# Autodesk Inventor assembly: 8022581 ESBF-BS-40-100-16P---(0)
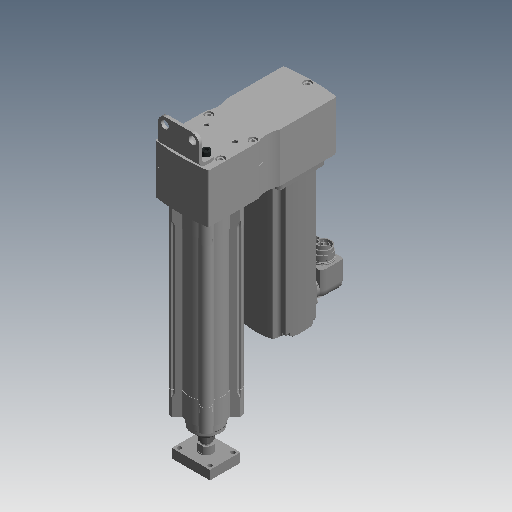
[picture p0: Inventor's stored thumbnail of the model, 512x512]
Saved by Autodesk Inventor 2021 (Build 250183000, 183)
## iProperties
Category: PARTsolutions
Company: FESTO
Part Number: 8022581 ESBF-BS-40-100-16P---(0)
Catalog Web Link: www.cadenas.de
Description: ESBF-Electro-cylinder
Vendor: FESTO
Document SubType Name: Assembly
Designer: partserver
Manufacturer: FESTO
Mass: 1707 g
Surface Area: 1273.02 cm^2
Volume: 500.946 cm^3
Density: 3.40756 g/cm^3
PSOL_IDENT_0: {ATYP=ASSISTANT},{DATA=script=$CADENAS_DATA/23d-libs/festo/webfesto.vbb&M_FAMILY=ESBF&M_GROUP=01&M_P
PSOL_IDENT_1: ARTNO=8022581&IDCODE1=ESBF-BS-40-100-16P&IDCODE2=&customer_number_cns=&MATES=1&LOD=HI&LOCKERP=0&SING
PSOL_IDENT_2: LEPART=1}
NB: 8022581 ESBF-BS-40-100-16P---(0)
NN: ESBF
NT: Electro-cylinder
NBSYN: $TNR. $TYP.---($HUBST.)
LINA: 8022581 ESBF-BS-40-100-16P
CATALOG: Festo
TNR: 8022581
TYP: ESBF-BS-40-100-16P
ANT: BS
KDM: 40
HUB: 100
SPI: 16P
HUBST: 0
AM: 24
WH: 29.5
L1: 14
L2: 244
L3: 18.4
L4: 14
L5: 3.3
L7: 24
L8: 4
G: 30
G1: 30
VA: 7
VD: 9
ZJ: 273.5
KK: M12x1.25
MM: 24
B: 39
D1: 24
D2: 8
D3: 40
BG: 16
EE: M7
E: 54
RT: M6
SW1: 13
SW2: 19
SW3: 6
TG: 38
CNSMASSEXACT: 1.707
SUPPLIER: FESTO
ARTICLENO: 8022581 ESBF-BS-40-100-16P---(0)
BOMINFO: 8022581 ESBF-BS-40-100-16P
CREATOR: CADENAS GmbH
Title: 8022581 ESBF-BS-40-100-16P
Author: Cadenas PARTsolutions
Comments: Electro-cylinder
## Documents named in this file (9)
- C:\Users\Santiago Suárez\Documents\GitHub\Dis.-Mecatronico-E6\Entrega Final\CAD\Mecanismo4dof\ActuadorAvance\AIS2021\8022581 ESBF-BS-40-100-16P---(0).iam
- C:\Users\Santiago Suárez\Documents\GitHub\Dis.-Mecatronico-E6\Entrega Final\CAD\Mecanismo4dof\ActuadorAvance\AIS2021\ESBF-BS-40-100---(ZR_-_-).ipt
- C:\Users\Santiago Suárez\Documents\GitHub\Dis.-Mecatronico-E6\Entrega Final\CAD\Mecanismo4dof\ActuadorAvance\AIS2021\ESBF-BS-40-100-5P---(KS_0).ipt
- C:\Users\Santiago Suárez\Documents\GitHub\Dis.-Mecatronico-E6\Entrega Final\CAD\Mecanismo4dof\ActuadorAvance\AIS2021\717739 GUK M10x0_75.ipt
- C:\Users\Santiago Suárez\Documents\GitHub\Dis.-Mecatronico-E6\Entrega Final\CAD\Mecanismo4dof\ActuadorAvance\AIS2021\ESBF-BS-40-ESBF-BS-40---(KSA).ipt
- C:\Users\Santiago Suárez\Documents\GitHub\Dis.-Mecatronico-E6\Entrega Final\CAD\Mecanismo4dof\ActuadorAvance\AIS2021\5242214 EMMT-AS-60-L-LS-RSB---(high).iam
- C:\Users\Santiago Suárez\Documents\GitHub\Dis.-Mecatronico-E6\Entrega Final\CAD\Mecanismo4dof\ActuadorAvance\36126 KSZ-M12x1,25.ipt
- C:\Users\Santiago Suárez\Documents\GitHub\Dis.-Mecatronico-E6\Entrega Final\CAD\Mecanismo4dof\ActuadorAvance\AIS2021\174370 HNC-40_(50).iam
- C:\Users\Santiago Suárez\Documents\GitHub\Dis.-Mecatronico-E6\Entrega Final\CAD\Mecanismo4dof\ActuadorAvance\AIS2021\2617488 EAMM-U-70-D40-60P-96.iam
## Components (8 placed, 8 different names)
1. ESBF-BS-40-100---(ZR_-_-):1 — KS_XY@1 <-> ANBAU_XY@2, KS_Z@1 <-> ANBAU_Z@2, KS_YZ@1 <-> ANBAU_YZ@2, GUA_XY@1 <-> ANBAU_XY@4, GUA_Z@1 <-> ANBAU_Z@4, GUA_YZ@1 <-> ANBAU_YZ@4, KSA_XY@1 <-> ANBAU_XY@5, KSA_Z@1 <-> ANBAU_Z@5, KSA_YZ@1 <-> ANBAU_YZ@5, Rigid:4
2. ESBF-BS-40-100-5P---(KS_0):1 — KS_XY@1 <-> ANBAU_XY@2, KS_Z@1 <-> ANBAU_Z@2, KS_YZ@1 <-> ANBAU_YZ@2, Rigid:2
3. 717739 GUK M10x0_75:1 — GUA_XY@1 <-> ANBAU_XY@4, GUA_Z@1 <-> ANBAU_Z@4, GUA_YZ@1 <-> ANBAU_YZ@4
4. ESBF-BS-40-ESBF-BS-40---(KSA):1 — KSA_XY@1 <-> ANBAU_XY@5, KSA_Z@1 <-> ANBAU_Z@5, KSA_YZ@1 <-> ANBAU_YZ@5
5. 5242214 EMMT-AS-60-L-LS-RSB---(high):1 [sub-assembly] — Rigid:3
6. 36126 KSZ-M12x1,25:1 — Rigid:2
7. 174370 HNC-40_(50):1 [sub-assembly] — Rigid:5
8. 2617488 EAMM-U-70-D40-60P-96:1 [sub-assembly] — Rigid:3, Rigid:4, Rigid:5
## Relationships (13: Mate 6, WeldJoint 4, Angle 3)
- KS_XY@1 <-> ANBAU_XY@2 [Mate]: ESBF-BS-40-100---(ZR_-_-):1 ↔ ESBF-BS-40-100-5P---(KS_0):1
- KS_Z@1 <-> ANBAU_Z@2 [Mate]: ESBF-BS-40-100---(ZR_-_-):1 ↔ ESBF-BS-40-100-5P---(KS_0):1
- KS_YZ@1 <-> ANBAU_YZ@2 [Angle] (0 deg): ESBF-BS-40-100---(ZR_-_-):1 ↔ ESBF-BS-40-100-5P---(KS_0):1
- GUA_XY@1 <-> ANBAU_XY@4 [Mate]: ESBF-BS-40-100---(ZR_-_-):1 ↔ 717739 GUK M10x0_75:1
- GUA_Z@1 <-> ANBAU_Z@4 [Mate]: ESBF-BS-40-100---(ZR_-_-):1 ↔ 717739 GUK M10x0_75:1
- GUA_YZ@1 <-> ANBAU_YZ@4 [Angle] (0 deg): ESBF-BS-40-100---(ZR_-_-):1 ↔ 717739 GUK M10x0_75:1
- KSA_XY@1 <-> ANBAU_XY@5 [Mate]: ESBF-BS-40-100---(ZR_-_-):1 ↔ ESBF-BS-40-ESBF-BS-40---(KSA):1
- KSA_Z@1 <-> ANBAU_Z@5 [Mate]: ESBF-BS-40-100---(ZR_-_-):1 ↔ ESBF-BS-40-ESBF-BS-40---(KSA):1
- KSA_YZ@1 <-> ANBAU_YZ@5 [Angle] (0 deg): ESBF-BS-40-100---(ZR_-_-):1 ↔ ESBF-BS-40-ESBF-BS-40---(KSA):1
- Rigid:2 [WeldJoint]: ESBF-BS-40-100-5P---(KS_0):1 ↔ 36126 KSZ-M12x1,25:1
- Rigid:3 [WeldJoint]: 5242214 EMMT-AS-60-L-LS-RSB---(high):1 ↔ 2617488 EAMM-U-70-D40-60P-96:1
- Rigid:4 [WeldJoint]: ESBF-BS-40-100---(ZR_-_-):1 ↔ 2617488 EAMM-U-70-D40-60P-96:1
- Rigid:5 [WeldJoint]: 174370 HNC-40_(50):1 ↔ 2617488 EAMM-U-70-D40-60P-96:1
